# Autodesk Inventor assembly: 12mmsmoothrod_CPY
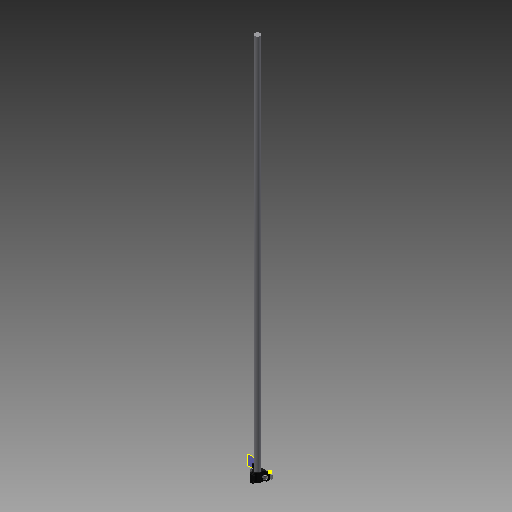
[picture p0: Inventor's stored thumbnail of the model, 512x512]
Saved by Autodesk Inventor 2017 (Build 210142000, 142)
## iProperties
Created: 2016-07-25
Part Number: 12mmsmoothrod_CPY
Document SubType Name: Assembly
Designer: User
Author: User
## Documents named in this file (5)
- C:\All INVENTOR\SL-Inventor\SL-Beast 3D Printer\12mmsmoothrod_CPY.iam
- C:\All INVENTOR\SL-Inventor\SL-Beast 3D Printer\12mmSmoothRod_CPY.ipt
- C:\All INVENTOR\SL-Inventor\SL-Beast 3D Printer\12mmrodholder_CPY.ipt
- C:\All INVENTOR\SL-Inventor\SL-Beast 3D Printer\en-US\ANSI B18.3.1M(6)\ANSI B18.3.1M - M5x0.8 x 10(1).ipt
- C:\All INVENTOR\SL-Inventor\SL-Beast 3D Printer\M5 Tee Nut-Generic_MIR_CPY_CPY.ipt
## Components (6 placed, 4 different names)
1. 12mmSmoothRod_CPY:1 — Mate:1
2. 12mmrodholder_CPY:1 — Mate:1, Insert:1, Insert:2
3. Forged Socket Head Cap Screw - Metric M5x0.8 x 10:1 — Insert:1, Mate:2
4. Forged Socket Head Cap Screw - Metric M5x0.8 x 10:2 — Insert:2, Mate:3
5. M5 Tee Nut-Generic_MIR_CPY_CPY:1 — Mate:2, Flush:1
6. M5 Tee Nut-Generic_MIR_CPY_CPY:2 — Mate:3, Flush:1
## Relationships (6: Mate 3, Insert 2, Flush 1)
- Mate:1: 12mmSmoothRod_CPY:1 ↔ 12mmrodholder_CPY:1
- Insert:1: 12mmrodholder_CPY:1 ↔ Forged Socket Head Cap Screw - Metric M5x0.8 x 10:1
- Insert:2: 12mmrodholder_CPY:1 ↔ Forged Socket Head Cap Screw - Metric M5x0.8 x 10:2
- Mate:2: Forged Socket Head Cap Screw - Metric M5x0.8 x 10:1 ↔ M5 Tee Nut-Generic_MIR_CPY_CPY:1
- Mate:3: Forged Socket Head Cap Screw - Metric M5x0.8 x 10:2 ↔ M5 Tee Nut-Generic_MIR_CPY_CPY:2
- Flush:1: M5 Tee Nut-Generic_MIR_CPY_CPY:1 ↔ M5 Tee Nut-Generic_MIR_CPY_CPY:2
